# Autodesk Inventor assembly: 00968-9015
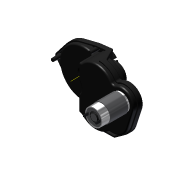
[picture p0: Inventor's stored thumbnail of the model, 180x180]
Saved by Autodesk Inventor 2011 SP1 (Build 150282100, 282)
## iProperties
Shininess: 64.0
Angle Display Precision: 2
Document Length Units: 11272
Document Angle Units: 11279
Document Time Units: 11290
Document Mass Units: 11286
Document Length Units Precision: 3
Document Angle Units Precision: 2
Category: Motors
Company: Autodesk, Inc.
Created: 2009-12-27
Document SubType Name: Assembly
Project: FIRST
Vendor: FisherPrice
Part Number: 00968-9015
Description: FisherPrice Motor and Gearbox
Catalog Web Link: www.fisher-price.com/powerwheels
Designer: Autodesk, Inc.
Density: 0.0
Volumn: 0.0
Area: 0.0
PropertySet Name: Model Information
Control State: 0
Master: False
Checked Out: False
Title: FisherPrice Motor and Gearbox
Author: Autodesk, Inc.
## Documents named in this file (4)
- D:\@vex2-for Upload\Motors\Motors_FisherPrice_00968-9015.iam
- D:\@vex2-for Upload\Motors\00968-9015_Housing2.ipt
- D:\@vex2-for Upload\Motors\00968-9015_Housing1.ipt
- D:\@vex2-for Upload\Motors\00968-9015_Spindle.ipt
## Components (3 placed, 3 different names)
1. 00968-9015_Housing2:1 — Flush:1, Flush:2, Mate:2, Mate:3
2. 00968-9015_Housing1:1 — Flush:1, Mate:1, Mate:2, Mate:3
3. 00968-9015_Spindle:1 — Flush:2, Mate:1
## Relationships (5: Mate 3, Flush 2)
- Flush:1: 00968-9015_Housing2:1 ↔ 00968-9015_Housing1:1
- Flush:2: 00968-9015_Housing2:1 ↔ 00968-9015_Spindle:1
- Mate:1: 00968-9015_Housing1:1 ↔ 00968-9015_Spindle:1
- Mate:2: 00968-9015_Housing2:1 ↔ 00968-9015_Housing1:1
- Mate:3: 00968-9015_Housing2:1 ↔ 00968-9015_Housing1:1
